# Autodesk Inventor assembly: KP_Semchuk
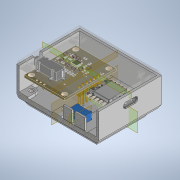
[picture p0: Inventor's stored thumbnail of the model, 180x180]
Saved by Autodesk Inventor 2021 (Build 250183000, 183)
## iProperties
Created: 2024-05-08
Part Number: KP_Semchuk
Document SubType Name: Assembly
Designer: Мария
Author: Мария
## Documents named in this file (8)
- D:\Documents\Inventor\Разводка печатных плат\KP_Semchuk.iam
- D:\Documents\Inventor\Разводка печатных плат\seeed-studio-xiao-esp32-c3-1.snapshot.8\Seeed Studio XIAO-ESP32-C3.ipt
- D:\Documents\Inventor\Разводка печатных плат\ad8232-2.snapshot.2\AD8232 v4.ipt
- D:\Documents\Inventor\Разводка печатных плат\seeed-studio-xiao-esp32-c3-1.snapshot.8\SW_DIP_SPSTx01_Slide_9.78x4.72mm_W7.62mm_P2.54mm.ipt
- D:\Documents\Inventor\Разводка печатных плат\крышка.ipt
- D:\Documents\Inventor\Разводка печатных плат\корпус.ipt
- D:\Documents\Inventor\Разводка печатных плат\Скоба.ipt
- D:\Documents\Inventor\Разводка печатных плат\движок.ipt
## Components (8 placed, 7 different names)
1. Seeed Studio XIAO-ESP32-C3:1
2. AD8232 v4:1
3. SW_DIP_SPSTx01_Slide_9.78x4.72mm_W7.62mm_P2.54mm:1
4. крышка:1 — Заподлицо:1, Заподлицо:2, Совмещение:9
5. корпус:1 — Заподлицо:1, Заподлицо:2, Совмещение:9, Угол:2, Совмещение:11, Совмещение:12, Совмещение:13, Заподлицо:5, Совмещение:14, Совмещение:16, Угол:3
6. Скоба:1 — Угол:2, Совмещение:11, Совмещение:12, Совмещение:13
7. SW_DIP_SPSTx01_Slide_9.78x4.72mm_W7.62mm_P2.54mm:2 — Заподлицо:5, Совмещение:14
8. движок:1 — Совмещение:16, Угол:3
## Relationships (11: Mate 6, Flush 3, Angle 2)
- Заподлицо:1 [Flush]: крышка:1 ↔ корпус:1
- Заподлицо:2 [Flush]: крышка:1 ↔ корпус:1
- Совмещение:9 [Mate]: крышка:1 ↔ корпус:1
- Угол:2 [Angle] (180 deg): корпус:1 ↔ Скоба:1
- Совмещение:11 [Mate]: корпус:1 ↔ Скоба:1
- Совмещение:12 [Mate]: корпус:1 ↔ Скоба:1
- Совмещение:13 [Mate]: корпус:1 ↔ Скоба:1
- Заподлицо:5 [Flush] (3.25 mm): корпус:1 ↔ SW_DIP_SPSTx01_Slide_9.78x4.72mm_W7.62mm_P2.54mm:2
- Совмещение:14 [Mate]: корпус:1 ↔ SW_DIP_SPSTx01_Slide_9.78x4.72mm_W7.62mm_P2.54mm:2
- Совмещение:16 [Mate]: корпус:1 ↔ движок:1
- Угол:3 [Angle] (0 deg): корпус:1 ↔ движок:1
